# Autodesk Inventor assembly: bumper_mirrored
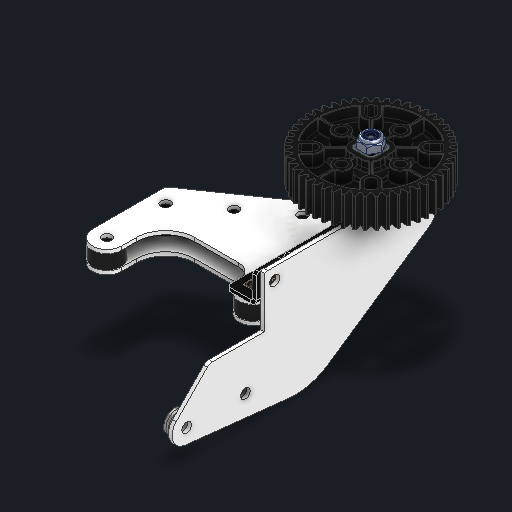
[picture p0: Inventor's stored thumbnail of the model, 512x512]
Saved by Autodesk Inventor 2024 (Build 280153000, 153)
## iProperties
Created: 2024-02-11
Part Number: bumper_mirrored
Document SubType Name: Assembly
Designer: Averey Ku
Author: Averey Ku
## Documents named in this file (15)
- D:\vex_robotics\hardware\cad\vroomba_v0.1\chassis\drivebay\mirrored_parts\bumper_mirrored.iam
- D:\vex_robotics\hardware\cad\vroomba_v0.1\chassis\drivebay\mirrored_parts\gusset_mirrored.ipt
- D:\vex_robotics\hardware\cad\VEX-CAD-Inventor-1.41\Motion\Spacers\Spacer Nylon .500 OD\NSpacer Black .500 OD x .250.ipt
- D:\vex_robotics\hardware\cad\VEX-CAD-Inventor-1.41\Motion\Spacers\Spacer Nylon .500 OD.ipt
- D:\vex_robotics\hardware\cad\vroomba_v0.1\chassis\drivebay\mirrored_parts\Alu Angle 1x1x6_mirrored.ipt
- D:\vex_robotics\hardware\cad\vroomba_v0.1\chassis\drivebay\mirrored_parts\Nut Keps_mirrored.ipt
- D:\vex_robotics\hardware\cad\VEX-CAD-Inventor-1.41\Motion\Spacers\Spacer Nylon .375 OD\NSpacer .375 OD x .375.ipt
- D:\vex_robotics\hardware\cad\VEX-CAD-Inventor-1.41\Motion\Spacers\Spacer Nylon .375 OD.ipt
- D:\vex_robotics\hardware\cad\vroomba_v0.1\chassis\drivebay\mirrored_parts\HS 48T Gear, No Insert_mirrored.iam
- D:\vex_robotics\hardware\cad\vroomba_v0.1\chassis\drivebay\mirrored_parts\Nut Thin Nylock_mirrored.ipt
- D:\vex_robotics\hardware\cad\vroomba_v0.1\chassis\drivebay\mirrored_parts\sled_mirrored.ipt
- D:\vex_robotics\hardware\cad\VEX-CAD-Inventor-1.41\Motion\Spacers\Washer Steel\SWasher .375 OD x .062500.ipt
- D:\vex_robotics\hardware\cad\VEX-CAD-Inventor-1.41\Motion\Spacers\Washer Steel.ipt
- D:\vex_robotics\hardware\cad\VEX-CAD-Inventor-1.41\Motion\Spacers\Washer Teflon\TWasher .375 OD x .04000.ipt
- D:\vex_robotics\hardware\cad\VEX-CAD-Inventor-1.41\Motion\Spacers\Washer Teflon.ipt
## Components (21 placed, 10 different names)
1. gusset_mirrored:1 — Insert:1, Insert:2, Insert:3, Insert:4, Insert:7, Insert:6, Insert:8
2. gusset_mirrored:2 — Mate:1, Insert:5, Mate:2, Insert:9
3. NSpacer Black .500 OD x .250:1 — Insert:1
4. NSpacer Black .500 OD x .250:2 — Insert:2
5. NSpacer Black .500 OD x .250:3 — Mate:1, Insert:3
6. NSpacer Black .500 OD x .250:4 — Insert:5, Insert:4
7. NSpacer Black .500 OD x .250:5 — Insert:7
8. NSpacer Black .500 OD x .250:6 — Insert:6
9. NSpacer Black .500 OD x .250:7 — Insert:8
10. Alu Angle 1x1x6_mirrored:1 — Mate:2, Insert:9, Insert:10, Mate:3, Insert:14
11. Nut Keps_mirrored:1 — Insert:10, Insert:11
12. NSpacer .375 OD x .375:1 — Insert:11, Insert:12
13. HS 48T Gear, No Insert_mirrored:1 [sub-assembly] — Insert:12, Insert:13
14. Nut Thin Nylock_mirrored:1 — Insert:13
15. sled_mirrored:1 — Mate:3, Insert:14, Insert:17, Insert:20
16. SWasher .375 OD x .062500:1 — Insert:17, Insert:16
17. TWasher .375 OD x .04000:1 — Insert:15
18. TWasher .375 OD x .04000:2 — Insert:16, Insert:15
19. SWasher .375 OD x .062500:2 — Insert:20, Insert:19
20. TWasher .375 OD x .04000:3 — Insert:18
21. TWasher .375 OD x .04000:4 — Insert:19, Insert:18
## Relationships (23: Insert 20, Mate 3)
- Insert:1: gusset_mirrored:1 ↔ NSpacer Black .500 OD x .250:1
- Insert:2: gusset_mirrored:1 ↔ NSpacer Black .500 OD x .250:2
- Mate:1: gusset_mirrored:2 ↔ NSpacer Black .500 OD x .250:3
- Insert:3: gusset_mirrored:1 ↔ NSpacer Black .500 OD x .250:3
- Insert:5: gusset_mirrored:2 ↔ NSpacer Black .500 OD x .250:4
- Insert:4: gusset_mirrored:1 ↔ NSpacer Black .500 OD x .250:4
- Insert:7: gusset_mirrored:1 ↔ NSpacer Black .500 OD x .250:5
- Insert:6: gusset_mirrored:1 ↔ NSpacer Black .500 OD x .250:6
- Insert:8: gusset_mirrored:1 ↔ NSpacer Black .500 OD x .250:7
- Mate:2: gusset_mirrored:2 ↔ Alu Angle 1x1x6_mirrored:1
- Insert:9: gusset_mirrored:2 ↔ Alu Angle 1x1x6_mirrored:1
- Insert:10: Alu Angle 1x1x6_mirrored:1 ↔ Nut Keps_mirrored:1
- Insert:11: Nut Keps_mirrored:1 ↔ NSpacer .375 OD x .375:1
- Insert:12: NSpacer .375 OD x .375:1 ↔ HS 48T Gear, No Insert_mirrored:1
- Insert:13: HS 48T Gear, No Insert_mirrored:1 ↔ Nut Thin Nylock_mirrored:1
- Mate:3: Alu Angle 1x1x6_mirrored:1 ↔ sled_mirrored:1
- Insert:14: Alu Angle 1x1x6_mirrored:1 ↔ sled_mirrored:1
- Insert:17: sled_mirrored:1 ↔ SWasher .375 OD x .062500:1
- Insert:16: SWasher .375 OD x .062500:1 ↔ TWasher .375 OD x .04000:2
- Insert:15: TWasher .375 OD x .04000:1 ↔ TWasher .375 OD x .04000:2
- Insert:20: sled_mirrored:1 ↔ SWasher .375 OD x .062500:2
- Insert:19: SWasher .375 OD x .062500:2 ↔ TWasher .375 OD x .04000:4
- Insert:18: TWasher .375 OD x .04000:3 ↔ TWasher .375 OD x .04000:4
